# Autodesk Inventor assembly: CNC3
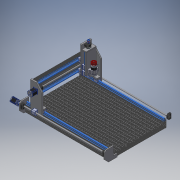
[picture p0: Inventor's stored thumbnail of the model, 180x180]
Saved by Autodesk Inventor 2018 (Build 220112000, 112)
## iProperties
Created: 2018-10-09
Part Number: CNC3
Material: Genérico
Document SubType Name: Assembly
Designer: Georgines
Author: Georgines
## Documents named in this file (29)
- C:\Users\Georgines\Documents\OpenCNC\MONTAGEM\CNC3.iam
- C:\Users\Georgines\Documents\OpenCNC\COMPONENTES_MECANICOS\BLOCOS_GUIAS_LINEARES\SBR16UU.ipt
- C:\Users\Georgines\Documents\OpenCNC\MONTAGEM\CNC1\APOIO_PERFIL_STRUTURAL.ipt
- C:\Users\Georgines\Documents\OpenCNC\MONTAGEM\CNC1\LATERAL_BLOCOS_BASE.ipt
- C:\Users\Georgines\Documents\OpenCNC\MONTAGEM\BLOCO_SUPORTE_EIXO_Z.ipt
- C:\Users\Georgines\Documents\OpenCNC\BAIXADOS\spindle-bldc-500w-1.snapshot.1\SPINDLE_500WSpindle.iam
- C:\Users\Georgines\Documents\OpenCNC\BAIXADOS\spindle-bracket-1.snapshot.2\SUPORTE_SPINDLESpindle Bracket.ipt
- C:\Users\Georgines\Documents\OpenCNC\MONTAGEM\CNC1\BLOCO_SUPORTE_SPINDLE.ipt
- C:\Users\Georgines\Documents\OpenCNC\BAIXADOS\bearing-support-unit-1.snapshot.1\BK12BK12.ipt
- C:\Users\Georgines\Documents\OpenCNC\BAIXADOS\bearing-support-unit-1.snapshot.1\BF12.ipt
- C:\Users\Georgines\Documents\OpenCNC\COMPONENTES_MECANICOS\GUIAS_LINEARES\SBR16_200MM.ipt
- C:\Users\Georgines\Documents\OpenCNC\COMPONENTES_MECANICOS\GUIAS_LINEARES\SBR16_EIXO_X_1.ipt
- C:\Users\Georgines\Documents\OpenCNC\BAIXADOS\stepper motor NEMA 23 57x76.ipt
- C:\Users\Georgines\Documents\OpenCNC\MONTAGEM\CHAPA_APOIO_CASTANHA_EIXO_Z.ipt
- C:\Users\Georgines\Documents\OpenCNC\COMPONENTES_MECANICOS\GUIAS_LINEARES\SBR16_EIXO_Y_1.ipt
- C:\Users\Georgines\Documents\OpenCNC\COMPONENTES_MECANICOS\GUIAS_LINEARES\SBR16_EIXO_Y_2.ipt
- C:\Users\Georgines\Documents\OpenCNC\COMPONENTES_MECANICOS\PERFIL_ESTRUTURAL\PERFIL_ESTRUTURAL_40X80_EIXO_Y.ipt
- C:\Users\Georgines\Documents\OpenCNC\COMPONENTES_MECANICOS\PERFIL_ESTRUTURAL\PERFIL_ESTRUTURAL_40X40_EIXO_Y_PERPENDICULAR.ipt
- C:\Users\Georgines\Documents\OpenCNC\COMPONENTES_MECANICOS\FUSOS\SFU16XX_Y1.ipt
- C:\Users\Georgines\Documents\OpenCNC\COMPONENTES_MECANICOS\FUSOS\SFU16XX_Y2.ipt
- C:\Users\Georgines\Documents\OpenCNC\COMPONENTES_MECANICOS\FUSOS\SFU16XX_Z.ipt
- C:\Users\Georgines\Documents\OpenCNC\COMPONENTES_MECANICOS\FUSOS\SFU16XX_X.ipt
- C:\Users\Georgines\Documents\OpenCNC\COMPONENTES_MECANICOS\CASTANHAS\CASTANHA_SFU1604SFU1604.ipt
- C:\Users\Georgines\Documents\OpenCNC\COMPONENTES_MECANICOS\ACOPLADORES\ACLOPLADOR_Jaw 6,35x10 d=25 L=30.ipt
- C:\Users\Georgines\Documents\OpenCNC\COMPONENTES_MECANICOS\PERFIL_ESTRUTURAL\PERFIL_ESTRUTURAL_30X60_EIXO_X1.ipt
- C:\Users\Georgines\Documents\OpenCNC\COMPONENTES_MECANICOS\PERFIL_ESTRUTURAL\PERFIL_ESTRUTURAL_30X60_EIXO_X2.ipt
- C:\Users\Georgines\Documents\OpenCNC\COMPONENTES_MECANICOS\SUPORTE_CASTANHAS\SUPORTE_CASTANHAS_DSG16H.ipt
- C:\Users\Georgines\Documents\OpenCNC\MONTAGEM\SUPORTE_MANCAL_FRONTAL.ipt
- C:\Users\Georgines\Documents\OpenCNC\COMPONENTES_MECANICOS\PERFIL_ESTRUTURAL\PERFIL_ESTRUTURAL_20X40_MESA.ipt
## Components (79 placed, 28 different names)
1. SBR16UU:1 — ALINHAMENTO_BOCOS_BASE, ALINHAMENTO_BOCOS_BASE_4, ALINHAMENTO_BOCOS_BASE_6, Alinhamento:32, Alinhamento:33, Coincidência:22, Coincidência:109
2. SBR16UU:2 — ALINHAMENTO_BOCOS_BASE_2, ALINHAMENTO_BOCOS_BASE_4, Alinhamento:31, Alinhamento:149, Coincidência:110
3. SBR16UU:3 — ALINHAMENTO_BOCOS_BASE_2, Alinhamento:81, Alinhamento:148, Coincidência:111
4. SBR16UU:4 — ALINHAMENTO_BOCOS_BASE, ALINHAMENTO_BOCOS_BASE_6, Coincidência:49, Alinhamento:82, Coincidência:108
5. APOIO_PERFIL_STRUTURAL:1 — Alinhamento:31, Alinhamento:32, Alinhamento:33, Coincidência:22, Coincidência:51, Alinhamento:85, Alinhamento:149, Alinhamento:177, Alinhamento:248
6. LATERAL_BLOCOS_BASE:1 — Alinhamento:83, Coincidência:51, Alinhamento:85, Alinhamento:177, Coincidência:173, Alinhamento:191, Alinhamento:192, Coincidência:191, Ângulo:3, Alinhamento:200, Ângulo:9, Coincidência:198, Ângulo:16, Alinhamento:208
7. BLOCO_SUPORTE_EIXO_Z:1 — Coincidência:66, Coincidência:77, Alinhamento:118, Alinhamento:122, Alinhamento:123, Alinhamento:124, Alinhamento:193, Coincidência:185, Coincidência:186, Alinhamento:196, Alinhamento:197, Coincidência:200, Alinhamento:202, Coincidência:204
8. APOIO_PERFIL_STRUTURAL:2 — Coincidência:49, Alinhamento:81, Alinhamento:82, Coincidência:52, Alinhamento:87, Alinhamento:148
9. LATERAL_BLOCOS_BASE:2 — Alinhamento:83, Coincidência:52, Alinhamento:87, Coincidência:174, Coincidência:194, Ângulo:4, Alinhamento:201, Ângulo:10, Coincidência:204
10. SPINDLE_500WSpindle:1 [sub-assembly] — Coincidência:63, Alinhamento:99
11. SUPORTE_SPINDLESpindle Bracket:1 — Coincidência:62, Alinhamento:97, Alinhamento:98, Coincidência:63, Alinhamento:99
12. BLOCO_SUPORTE_SPINDLE:1 — Coincidência:62, Alinhamento:97, Alinhamento:98, Coincidência:79, Coincidência:81, Alinhamento:119, Alinhamento:120, Alinhamento:121, Alinhamento:151, Alinhamento:152, Alinhamento:153
13. BK12BK12:1 — Coincidência:66, Alinhamento:103, Alinhamento:124, Coincidência:181, Coincidência:182, Coincidência:203
14. BF12:1 — Alinhamento:103, Alinhamento:123, Coincidência:180, Coincidência:184
15. SBR16UU:9 — Alinhamento:104, Alinhamento:106, Alinhamento:109, Coincidência:75, Coincidência:76, Coincidência:77, Coincidência:78, Alinhamento:122
16. SBR16UU:10 — Alinhamento:104, Alinhamento:107, Alinhamento:108, Alinhamento:109, Coincidência:76, Coincidência:80
17. SBR16UU:11 — Alinhamento:105, Alinhamento:106, Alinhamento:110, Coincidência:75
18. SBR16UU:12 — Alinhamento:105, Alinhamento:107, Alinhamento:108, Alinhamento:110, Alinhamento:118
19. SBR16_200MM:1 — Coincidência:78, Coincidência:79, Alinhamento:119, Alinhamento:121
20. SBR16_200MM:2 — Coincidência:80, Coincidência:81, Alinhamento:120
21. SBR16UU:13 — Coincidência:169, Alinhamento:189, Alinhamento:194, Coincidência:186, Alinhamento:197
22. SBR16UU:14 — Coincidência:168, Alinhamento:190, Alinhamento:195, Coincidência:185, Alinhamento:196
23. SBR16UU:15 — Alinhamento:173, Coincidência:166, Alinhamento:190, Alinhamento:193, Alinhamento:195
24. stepper motor NEMA 23 57x76:1 — Coincidência:187, Coincidência:188, Coincidência:198, Ângulo:12
25. CHAPA_APOIO_CASTANHA_EIXO_Z:1 — Alinhamento:151, Alinhamento:152, Alinhamento:153, Coincidência:177, Ângulo:1
26. SBR16_EIXO_Y_1:1 — Coincidência:109, Coincidência:110, Alinhamento:154, Alinhamento:157, Coincidência:115, Alinhamento:158, Alinhamento:159
27. SBR16_EIXO_Y_2:1 — Coincidência:108, Coincidência:111, Alinhamento:154, Alinhamento:157, Coincidência:116, Alinhamento:160, Alinhamento:161
28. PERFIL_ESTRUTURAL_40X80_EIXO_Y:1 — Coincidência:115, Alinhamento:158, Alinhamento:159, Alinhamento:164, Alinhamento:165, Alinhamento:166, Coincidência:131, Coincidência:133, Ângulo:9, Alinhamento:203, Alinhamento:205
29. PERFIL_ESTRUTURAL_40X80_EIXO_Y:2 — Coincidência:116, Alinhamento:160, Alinhamento:161, Coincidência:117, Alinhamento:162, Alinhamento:163, Coincidência:118, Coincidência:119, Coincidência:132, Ângulo:10, Coincidência:231
30. PERFIL_ESTRUTURAL_40X40_EIXO_Y_PERPENDICULAR:1 — Coincidência:117, Alinhamento:162, Alinhamento:163, Coincidência:210, Alinhamento:247
31. PERFIL_ESTRUTURAL_40X40_EIXO_Y_PERPENDICULAR:2 — Coincidência:118, Alinhamento:164, Alinhamento:165, Alinhamento:167
32. PERFIL_ESTRUTURAL_40X40_EIXO_Y_PERPENDICULAR:3 — Coincidência:119, Alinhamento:166, Alinhamento:167
33. stepper motor NEMA 23 57x76:3 — Coincidência:159, Coincidência:160, Ângulo:17, Ângulo:18
34. SBR16UU:17 — Alinhamento:173, Coincidência:167, Alinhamento:189, Alinhamento:194
35. SFU16XX_Y1:1 — Coincidência:136, Coincidência:137, Coincidência:138, Coincidência:139, Coincidência:152, Coincidência:155, Coincidência:157
36. SFU16XX_Y2:1 — Coincidência:140, Coincidência:141, Coincidência:142, Coincidência:143, Coincidência:153, Coincidência:156, Coincidência:158
37. SFU16XX_Z:1 — Coincidência:178, Coincidência:179, Coincidência:180, Coincidência:181, Coincidência:182, Coincidência:183, Coincidência:184
38. SFU16XX_X:1 — Coincidência:146, Coincidência:148, Coincidência:149, Coincidência:151, Coincidência:154, Coincidência:175, Coincidência:176
39. BK12BK12:2 — Coincidência:136, Coincidência:137, Alinhamento:178, Ângulo:16, Coincidência:206
40. BF12:2 — Coincidência:138, Coincidência:139, Alinhamento:178, Alinhamento:181, Alinhamento:198, Alinhamento:203, Coincidência:205
41. BK12BK12:3 — Coincidência:140, Coincidência:141, Alinhamento:179
42. BF12:3 — Coincidência:142, Coincidência:143, Alinhamento:179, Alinhamento:181, Alinhamento:198
43. BK12BK12:4 — Coincidência:146, Alinhamento:180, Coincidência:151, Ângulo:12
44. BF12:4 — Coincidência:148, Coincidência:149, Alinhamento:180, Ângulo:14, Alinhamento:212
45. CASTANHA_SFU1604SFU1604:1 — Coincidência:152, Coincidência:189, Coincidência:190, Ângulo:2
46. CASTANHA_SFU1604SFU1604:2 — Coincidência:153, Coincidência:192, Coincidência:193, Ângulo:13
47. CASTANHA_SFU1604SFU1604:3 — Coincidência:154, Coincidência:195, Coincidência:196, Ângulo:11
48. CASTANHA_SFU1604SFU1604:4 — Coincidência:177, Coincidência:178, Ângulo:1, Coincidência:203
49. ACLOPLADOR_Jaw 6,35x10 d=25 L=30:1 — Coincidência:156, Coincidência:158, Coincidência:201, Coincidência:202
50. ACLOPLADOR_Jaw 6,35x10 d=25 L=30:2 — Coincidência:155, Coincidência:157, Coincidência:159, Coincidência:160
51. ACLOPLADOR_Jaw 6,35x10 d=25 L=30:3 — Coincidência:179, Coincidência:183
52. ACLOPLADOR_Jaw 6,35x10 d=25 L=30:4 — Coincidência:175, Coincidência:176, Coincidência:187, Coincidência:188
53. PERFIL_ESTRUTURAL_30X60_EIXO_X1:1 — Coincidência:163, Alinhamento:183, Alinhamento:184, Alinhamento:187, Alinhamento:188, Coincidência:173, Alinhamento:191, Coincidência:174, Alinhamento:192, Coincidência:207, Alinhamento:209, Alinhamento:210
54. PERFIL_ESTRUTURAL_30X60_EIXO_X2:1 — Coincidência:164, Alinhamento:185, Alinhamento:186, Alinhamento:187, Alinhamento:188, Coincidência:208, Alinhamento:211
55. SBR16_EIXO_X_1:2 — Coincidência:163, Alinhamento:183, Alinhamento:184, Coincidência:168, Coincidência:169, Ângulo:14
56. SBR16_EIXO_X_1:3 — Coincidência:164, Alinhamento:185, Alinhamento:186, Coincidência:166, Coincidência:167
57. SUPORTE_CASTANHAS_DSG16H:1 — Coincidência:189, Coincidência:190, Ângulo:2, Coincidência:191, Ângulo:3, Alinhamento:200, Coincidência:205, Alinhamento:208
58. SUPORTE_CASTANHAS_DSG16H:2 — Coincidência:192, Coincidência:193, Coincidência:194, Ângulo:4, Alinhamento:201, Ângulo:13
59. SUPORTE_CASTANHAS_DSG16H:3 — Coincidência:195, Coincidência:196, Ângulo:11, Coincidência:200, Alinhamento:202
60. stepper motor NEMA 23 57x76:4 — Coincidência:201, Coincidência:202, Ângulo:17
61. SUPORTE_MANCAL_FRONTAL:1 — Alinhamento:205, Alinhamento:206, Alinhamento:207, Coincidência:211, Alinhamento:247, Alinhamento:248
62. SUPORTE_MANCAL_FRONTAL:2 — Coincidência:206, Alinhamento:206, Alinhamento:207, Ângulo:18
63. PERFIL_ESTRUTURAL_30X60_EIXO_X1:2 — Coincidência:207, Alinhamento:209, Alinhamento:210, Coincidência:208, Alinhamento:211, Alinhamento:212
64. PERFIL_ESTRUTURAL_20X40_MESA:1 — Coincidência:209, Coincidência:210, Coincidência:211, Alinhamento:213, Alinhamento:214
65. PERFIL_ESTRUTURAL_20X40_MESA:2 — Coincidência:209, Alinhamento:213, Alinhamento:214, Alinhamento:215, Alinhamento:216, Coincidência:213
66. PERFIL_ESTRUTURAL_20X40_MESA:3 — Alinhamento:215, Alinhamento:216, Coincidência:213, Coincidência:214, Alinhamento:217, Alinhamento:218
67. PERFIL_ESTRUTURAL_20X40_MESA:4 — Coincidência:214, Coincidência:215, Alinhamento:217, Alinhamento:218, Coincidência:216, Alinhamento:219, Alinhamento:220
68. PERFIL_ESTRUTURAL_20X40_MESA:5 — Coincidência:215, Coincidência:216, Alinhamento:219, Alinhamento:220, Coincidência:217, Alinhamento:221, Alinhamento:222
69. PERFIL_ESTRUTURAL_20X40_MESA:6 — Coincidência:217, Alinhamento:221, Alinhamento:222, Coincidência:218, Alinhamento:223, Alinhamento:224
70. PERFIL_ESTRUTURAL_20X40_MESA:7 — Coincidência:218, Alinhamento:223, Alinhamento:224, Coincidência:219, Alinhamento:225, Alinhamento:226
71. PERFIL_ESTRUTURAL_20X40_MESA:8 — Coincidência:219, Alinhamento:225, Alinhamento:226, Coincidência:220, Alinhamento:227, Alinhamento:228
72. PERFIL_ESTRUTURAL_20X40_MESA:9 — Coincidência:220, Alinhamento:227, Alinhamento:228, Coincidência:230, Alinhamento:245, Alinhamento:246
73. PERFIL_ESTRUTURAL_20X40_MESA:10 — Coincidência:230, Alinhamento:245, Alinhamento:246
74. PERFIL_ESTRUTURAL_20X40_MESA:11
75. PERFIL_ESTRUTURAL_20X40_MESA:12
76. PERFIL_ESTRUTURAL_20X40_MESA:13
77. PERFIL_ESTRUTURAL_20X40_MESA:14
78. PERFIL_ESTRUTURAL_20X40_MESA:15
79. PERFIL_ESTRUTURAL_20X40_MESA:16 — Coincidência:231
## Relationships (233: Flush 113, Mate 107, Angle 13)
- ALINHAMENTO_BOCOS_BASE [Flush]: SBR16UU:1 ↔ SBR16UU:4
- ALINHAMENTO_BOCOS_BASE_2 [Flush]: SBR16UU:2 ↔ SBR16UU:3
- ALINHAMENTO_BOCOS_BASE_4 [Flush]: SBR16UU:1 ↔ SBR16UU:2
- ALINHAMENTO_BOCOS_BASE_6 [Flush]: SBR16UU:1 ↔ SBR16UU:4
- Alinhamento:31 [Flush]: SBR16UU:2 ↔ APOIO_PERFIL_STRUTURAL:1
- Alinhamento:32 [Flush]: SBR16UU:1 ↔ APOIO_PERFIL_STRUTURAL:1
- Alinhamento:33 [Flush]: SBR16UU:1 ↔ APOIO_PERFIL_STRUTURAL:1
- Coincidência:22 [Mate]: SBR16UU:1 ↔ APOIO_PERFIL_STRUTURAL:1
- Coincidência:49 [Mate]: SBR16UU:4 ↔ APOIO_PERFIL_STRUTURAL:2
- Alinhamento:81 [Flush]: SBR16UU:3 ↔ APOIO_PERFIL_STRUTURAL:2
- Alinhamento:82 [Flush]: SBR16UU:4 ↔ APOIO_PERFIL_STRUTURAL:2
- Alinhamento:83 [Flush]: LATERAL_BLOCOS_BASE:1 ↔ LATERAL_BLOCOS_BASE:2
- Coincidência:51 [Mate]: APOIO_PERFIL_STRUTURAL:1 ↔ LATERAL_BLOCOS_BASE:1
- Alinhamento:85 [Flush] (-55 mm): APOIO_PERFIL_STRUTURAL:1 ↔ LATERAL_BLOCOS_BASE:1
- Coincidência:52 [Mate]: APOIO_PERFIL_STRUTURAL:2 ↔ LATERAL_BLOCOS_BASE:2
- Alinhamento:87 [Flush]: APOIO_PERFIL_STRUTURAL:2 ↔ LATERAL_BLOCOS_BASE:2
- Coincidência:62 [Mate]: SUPORTE_SPINDLESpindle Bracket:1 ↔ BLOCO_SUPORTE_SPINDLE:1
- Alinhamento:97 [Flush] (25 mm): SUPORTE_SPINDLESpindle Bracket:1 ↔ BLOCO_SUPORTE_SPINDLE:1
- Alinhamento:98 [Flush] (18 mm): SUPORTE_SPINDLESpindle Bracket:1 ↔ BLOCO_SUPORTE_SPINDLE:1
- Coincidência:63 [Mate]: SPINDLE_500WSpindle:1 ↔ SUPORTE_SPINDLESpindle Bracket:1
- Alinhamento:99 [Flush] (-25 mm): SPINDLE_500WSpindle:1 ↔ SUPORTE_SPINDLESpindle Bracket:1
- Coincidência:66 [Mate]: BLOCO_SUPORTE_EIXO_Z:1 ↔ BK12BK12:1
- Alinhamento:103 [Flush]: BK12BK12:1 ↔ BF12:1
- Alinhamento:104 [Flush]: SBR16UU:9 ↔ SBR16UU:10
- Alinhamento:105 [Flush]: SBR16UU:11 ↔ SBR16UU:12
- Alinhamento:106 [Flush]: SBR16UU:9 ↔ SBR16UU:11
- Alinhamento:107 [Flush]: SBR16UU:10 ↔ SBR16UU:12
- Alinhamento:108 [Flush]: SBR16UU:10 ↔ SBR16UU:12
- Alinhamento:109 [Flush]: SBR16UU:9 ↔ SBR16UU:10
- Alinhamento:110 [Flush]: SBR16UU:11 ↔ SBR16UU:12
- Coincidência:75 [Mate] (23 mm): SBR16UU:9 ↔ SBR16UU:11
- Coincidência:76 [Mate] (35 mm): SBR16UU:9 ↔ SBR16UU:10
- Coincidência:77 [Mate]: BLOCO_SUPORTE_EIXO_Z:1 ↔ SBR16UU:9
- Alinhamento:118 [Flush]: BLOCO_SUPORTE_EIXO_Z:1 ↔ SBR16UU:12
- Coincidência:78 [Mate]: SBR16UU:9 ↔ SBR16_200MM:1
- Coincidência:79 [Mate]: BLOCO_SUPORTE_SPINDLE:1 ↔ SBR16_200MM:1
- Coincidência:80 [Mate]: SBR16UU:10 ↔ SBR16_200MM:2
- Coincidência:81 [Mate]: BLOCO_SUPORTE_SPINDLE:1 ↔ SBR16_200MM:2
- Alinhamento:119 [Flush]: BLOCO_SUPORTE_SPINDLE:1 ↔ SBR16_200MM:1
- Alinhamento:120 [Flush]: BLOCO_SUPORTE_SPINDLE:1 ↔ SBR16_200MM:2
- Alinhamento:121 [Flush] (-2.5 mm): BLOCO_SUPORTE_SPINDLE:1 ↔ SBR16_200MM:1
- Alinhamento:122 [Flush]: BLOCO_SUPORTE_EIXO_Z:1 ↔ SBR16UU:9
- Alinhamento:123 [Flush] (46.627 mm): BLOCO_SUPORTE_EIXO_Z:1 ↔ BF12:1
- Alinhamento:124 [Flush] (32.5 mm): BLOCO_SUPORTE_EIXO_Z:1 ↔ BK12BK12:1
- Alinhamento:148 [Flush]: SBR16UU:3 ↔ APOIO_PERFIL_STRUTURAL:2
- Alinhamento:149 [Flush]: SBR16UU:2 ↔ APOIO_PERFIL_STRUTURAL:1
- Alinhamento:151 [Flush]: BLOCO_SUPORTE_SPINDLE:1 ↔ CHAPA_APOIO_CASTANHA_EIXO_Z:1
- Alinhamento:152 [Flush]: BLOCO_SUPORTE_SPINDLE:1 ↔ CHAPA_APOIO_CASTANHA_EIXO_Z:1
- Alinhamento:153 [Flush]: BLOCO_SUPORTE_SPINDLE:1 ↔ CHAPA_APOIO_CASTANHA_EIXO_Z:1
- Coincidência:108 [Mate]: SBR16UU:4 ↔ SBR16_EIXO_Y_2:1
- Coincidência:109 [Mate]: SBR16UU:1 ↔ SBR16_EIXO_Y_1:1
- Coincidência:110 [Mate]: SBR16UU:2 ↔ SBR16_EIXO_Y_1:1
- Coincidência:111 [Mate]: SBR16UU:3 ↔ SBR16_EIXO_Y_2:1
- Alinhamento:154 [Flush]: SBR16_EIXO_Y_1:1 ↔ SBR16_EIXO_Y_2:1
- Alinhamento:157 [Flush]: SBR16_EIXO_Y_1:1 ↔ SBR16_EIXO_Y_2:1
- Coincidência:115 [Mate]: SBR16_EIXO_Y_1:1 ↔ PERFIL_ESTRUTURAL_40X80_EIXO_Y:1
- Coincidência:116 [Mate]: SBR16_EIXO_Y_2:1 ↔ PERFIL_ESTRUTURAL_40X80_EIXO_Y:2
- Alinhamento:158 [Flush]: SBR16_EIXO_Y_1:1 ↔ PERFIL_ESTRUTURAL_40X80_EIXO_Y:1
- Alinhamento:159 [Flush]: SBR16_EIXO_Y_1:1 ↔ PERFIL_ESTRUTURAL_40X80_EIXO_Y:1
- Alinhamento:160 [Flush]: SBR16_EIXO_Y_2:1 ↔ PERFIL_ESTRUTURAL_40X80_EIXO_Y:2
- Alinhamento:161 [Flush]: SBR16_EIXO_Y_2:1 ↔ PERFIL_ESTRUTURAL_40X80_EIXO_Y:2
- Coincidência:117 [Mate]: PERFIL_ESTRUTURAL_40X80_EIXO_Y:2 ↔ PERFIL_ESTRUTURAL_40X40_EIXO_Y_PERPENDICULAR:1
- Alinhamento:162 [Flush]: PERFIL_ESTRUTURAL_40X80_EIXO_Y:2 ↔ PERFIL_ESTRUTURAL_40X40_EIXO_Y_PERPENDICULAR:1
- Alinhamento:163 [Flush]: PERFIL_ESTRUTURAL_40X80_EIXO_Y:2 ↔ PERFIL_ESTRUTURAL_40X40_EIXO_Y_PERPENDICULAR:1
- Coincidência:118 [Mate]: PERFIL_ESTRUTURAL_40X80_EIXO_Y:2 ↔ PERFIL_ESTRUTURAL_40X40_EIXO_Y_PERPENDICULAR:2
- Alinhamento:164 [Flush]: PERFIL_ESTRUTURAL_40X80_EIXO_Y:1 ↔ PERFIL_ESTRUTURAL_40X40_EIXO_Y_PERPENDICULAR:2
- Alinhamento:165 [Flush]: PERFIL_ESTRUTURAL_40X80_EIXO_Y:1 ↔ PERFIL_ESTRUTURAL_40X40_EIXO_Y_PERPENDICULAR:2
- Coincidência:119 [Mate]: PERFIL_ESTRUTURAL_40X80_EIXO_Y:2 ↔ PERFIL_ESTRUTURAL_40X40_EIXO_Y_PERPENDICULAR:3
- Alinhamento:166 [Flush]: PERFIL_ESTRUTURAL_40X80_EIXO_Y:1 ↔ PERFIL_ESTRUTURAL_40X40_EIXO_Y_PERPENDICULAR:3
- Alinhamento:167 [Flush] (-433.419 mm): PERFIL_ESTRUTURAL_40X40_EIXO_Y_PERPENDICULAR:2 ↔ PERFIL_ESTRUTURAL_40X40_EIXO_Y_PERPENDICULAR:3
- Alinhamento:173 [Flush]: SBR16UU:15 ↔ SBR16UU:17
- Coincidência:131 [Mate]: PERFIL_ESTRUTURAL_40X80_EIXO_Y:1
- Coincidência:132 [Mate]: PERFIL_ESTRUTURAL_40X80_EIXO_Y:2
- Coincidência:133 [Mate]: PERFIL_ESTRUTURAL_40X80_EIXO_Y:1
- Alinhamento:177 [Flush]: APOIO_PERFIL_STRUTURAL:1 ↔ LATERAL_BLOCOS_BASE:1
- Coincidência:136 [Mate]: SFU16XX_Y1:1 ↔ BK12BK12:2
- Coincidência:137 [Mate]: SFU16XX_Y1:1 ↔ BK12BK12:2
- Coincidência:138 [Mate]: SFU16XX_Y1:1 ↔ BF12:2
- Coincidência:139 [Mate]: SFU16XX_Y1:1 ↔ BF12:2
- Coincidência:140 [Mate]: SFU16XX_Y2:1 ↔ BK12BK12:3
- Coincidência:141 [Mate]: SFU16XX_Y2:1 ↔ BK12BK12:3
- Coincidência:142 [Mate]: SFU16XX_Y2:1 ↔ BF12:3
- Coincidência:143 [Mate]: SFU16XX_Y2:1 ↔ BF12:3
- Alinhamento:178 [Flush]: BK12BK12:2 ↔ BF12:2
- Alinhamento:179 [Flush]: BK12BK12:3 ↔ BF12:3
- Coincidência:146 [Mate]: SFU16XX_X:1 ↔ BK12BK12:4
- Coincidência:148 [Mate]: SFU16XX_X:1 ↔ BF12:4
- Coincidência:149 [Mate]: SFU16XX_X:1 ↔ BF12:4
- Alinhamento:180 [Flush]: BK12BK12:4 ↔ BF12:4
- Coincidência:151 [Mate]: SFU16XX_X:1 ↔ BK12BK12:4
- Coincidência:152 [Mate]: SFU16XX_Y1:1 ↔ CASTANHA_SFU1604SFU1604:1
- Coincidência:153 [Mate]: SFU16XX_Y2:1 ↔ CASTANHA_SFU1604SFU1604:2
- Coincidência:154 [Mate]: SFU16XX_X:1 ↔ CASTANHA_SFU1604SFU1604:3
- Coincidência:155 [Mate]: SFU16XX_Y1:1 ↔ ACLOPLADOR_Jaw 6,35x10 d=25 L=30:2
- Coincidência:156 [Mate]: SFU16XX_Y2:1 ↔ ACLOPLADOR_Jaw 6,35x10 d=25 L=30:1
- Coincidência:157 [Mate]: SFU16XX_Y1:1 ↔ ACLOPLADOR_Jaw 6,35x10 d=25 L=30:2
- Coincidência:158 [Mate]: SFU16XX_Y2:1 ↔ ACLOPLADOR_Jaw 6,35x10 d=25 L=30:1
- Alinhamento:181 [Flush]: BF12:2 ↔ BF12:3
- Coincidência:159 [Mate]: stepper motor NEMA 23 57x76:3 ↔ ACLOPLADOR_Jaw 6,35x10 d=25 L=30:2
- Coincidência:160 [Mate] (-15 mm): stepper motor NEMA 23 57x76:3 ↔ ACLOPLADOR_Jaw 6,35x10 d=25 L=30:2
- Coincidência:163 [Mate]: PERFIL_ESTRUTURAL_30X60_EIXO_X1:1 ↔ SBR16_EIXO_X_1:2
- Alinhamento:183 [Flush]: PERFIL_ESTRUTURAL_30X60_EIXO_X1:1 ↔ SBR16_EIXO_X_1:2
- Alinhamento:184 [Flush] (-10 mm): PERFIL_ESTRUTURAL_30X60_EIXO_X1:1 ↔ SBR16_EIXO_X_1:2
- Coincidência:164 [Mate]: PERFIL_ESTRUTURAL_30X60_EIXO_X2:1 ↔ SBR16_EIXO_X_1:3
- Alinhamento:185 [Flush]: PERFIL_ESTRUTURAL_30X60_EIXO_X2:1 ↔ SBR16_EIXO_X_1:3
- Alinhamento:186 [Flush] (10 mm): PERFIL_ESTRUTURAL_30X60_EIXO_X2:1 ↔ SBR16_EIXO_X_1:3
- Alinhamento:187 [Flush]: PERFIL_ESTRUTURAL_30X60_EIXO_X1:1 ↔ PERFIL_ESTRUTURAL_30X60_EIXO_X2:1
- Alinhamento:188 [Flush]: PERFIL_ESTRUTURAL_30X60_EIXO_X1:1 ↔ PERFIL_ESTRUTURAL_30X60_EIXO_X2:1
- Coincidência:166 [Mate]: SBR16UU:15 ↔ SBR16_EIXO_X_1:3
- Coincidência:167 [Mate]: SBR16UU:17 ↔ SBR16_EIXO_X_1:3
- Coincidência:168 [Mate]: SBR16UU:14 ↔ SBR16_EIXO_X_1:2
- Coincidência:169 [Mate]: SBR16UU:13 ↔ SBR16_EIXO_X_1:2
- Alinhamento:189 [Flush]: SBR16UU:13 ↔ SBR16UU:17
- Alinhamento:190 [Flush]: SBR16UU:14 ↔ SBR16UU:15
- Coincidência:173 [Mate]: LATERAL_BLOCOS_BASE:1 ↔ PERFIL_ESTRUTURAL_30X60_EIXO_X1:1
- Alinhamento:191 [Flush] (10 mm): LATERAL_BLOCOS_BASE:1 ↔ PERFIL_ESTRUTURAL_30X60_EIXO_X1:1
- Coincidência:174 [Mate]: LATERAL_BLOCOS_BASE:2 ↔ PERFIL_ESTRUTURAL_30X60_EIXO_X1:1
- Alinhamento:192 [Flush]: LATERAL_BLOCOS_BASE:1 ↔ PERFIL_ESTRUTURAL_30X60_EIXO_X1:1
- Alinhamento:193 [Flush]: BLOCO_SUPORTE_EIXO_Z:1 ↔ SBR16UU:15
- Coincidência:175 [Mate]: SFU16XX_X:1 ↔ ACLOPLADOR_Jaw 6,35x10 d=25 L=30:4
- Coincidência:176 [Mate] (-15 mm): SFU16XX_X:1 ↔ ACLOPLADOR_Jaw 6,35x10 d=25 L=30:4
- Coincidência:177 [Mate]: CHAPA_APOIO_CASTANHA_EIXO_Z:1 ↔ CASTANHA_SFU1604SFU1604:4
- Coincidência:178 [Mate]: SFU16XX_Z:1 ↔ CASTANHA_SFU1604SFU1604:4
- Coincidência:179 [Mate]: SFU16XX_Z:1 ↔ ACLOPLADOR_Jaw 6,35x10 d=25 L=30:3
- Coincidência:180 [Mate]: BF12:1 ↔ SFU16XX_Z:1
- Coincidência:181 [Mate]: BK12BK12:1 ↔ SFU16XX_Z:1
- Coincidência:182 [Mate]: BK12BK12:1 ↔ SFU16XX_Z:1
- Ângulo:1 [Angle] (0 deg): CHAPA_APOIO_CASTANHA_EIXO_Z:1 ↔ CASTANHA_SFU1604SFU1604:4
- Coincidência:183 [Mate] (-15 mm): SFU16XX_Z:1 ↔ ACLOPLADOR_Jaw 6,35x10 d=25 L=30:3
- Coincidência:184 [Mate]: BF12:1 ↔ SFU16XX_Z:1
- Alinhamento:194 [Flush]: SBR16UU:13 ↔ SBR16UU:17
- Alinhamento:195 [Flush]: SBR16UU:14 ↔ SBR16UU:15
- Coincidência:185 [Mate]: BLOCO_SUPORTE_EIXO_Z:1 ↔ SBR16UU:14
- Coincidência:186 [Mate]: BLOCO_SUPORTE_EIXO_Z:1 ↔ SBR16UU:13
- Alinhamento:196 [Flush]: BLOCO_SUPORTE_EIXO_Z:1 ↔ SBR16UU:14
- Alinhamento:197 [Flush]: BLOCO_SUPORTE_EIXO_Z:1 ↔ SBR16UU:13
- Coincidência:187 [Mate]: stepper motor NEMA 23 57x76:1 ↔ ACLOPLADOR_Jaw 6,35x10 d=25 L=30:4
- Coincidência:188 [Mate] (-15 mm): stepper motor NEMA 23 57x76:1 ↔ ACLOPLADOR_Jaw 6,35x10 d=25 L=30:4
- Alinhamento:198 [Flush]: BF12:2 ↔ BF12:3
- Coincidência:189 [Mate]: CASTANHA_SFU1604SFU1604:1 ↔ SUPORTE_CASTANHAS_DSG16H:1
- Coincidência:190 [Mate]: CASTANHA_SFU1604SFU1604:1 ↔ SUPORTE_CASTANHAS_DSG16H:1
- Ângulo:2 [Angle] (0 deg): CASTANHA_SFU1604SFU1604:1 ↔ SUPORTE_CASTANHAS_DSG16H:1
- Coincidência:191 [Mate]: LATERAL_BLOCOS_BASE:1 ↔ SUPORTE_CASTANHAS_DSG16H:1
- Ângulo:3 [Angle] (0 deg): LATERAL_BLOCOS_BASE:1 ↔ SUPORTE_CASTANHAS_DSG16H:1
- Coincidência:192 [Mate]: CASTANHA_SFU1604SFU1604:2 ↔ SUPORTE_CASTANHAS_DSG16H:2
- Coincidência:193 [Mate]: CASTANHA_SFU1604SFU1604:2 ↔ SUPORTE_CASTANHAS_DSG16H:2
- Coincidência:194 [Mate]: LATERAL_BLOCOS_BASE:2 ↔ SUPORTE_CASTANHAS_DSG16H:2
- Ângulo:4 [Angle] (0 deg): LATERAL_BLOCOS_BASE:2 ↔ SUPORTE_CASTANHAS_DSG16H:2
- Alinhamento:200 [Flush] (-50 mm): LATERAL_BLOCOS_BASE:1 ↔ SUPORTE_CASTANHAS_DSG16H:1
- Alinhamento:201 [Flush] (50 mm): LATERAL_BLOCOS_BASE:2 ↔ SUPORTE_CASTANHAS_DSG16H:2
- Ângulo:9 [Angle] (0 deg): LATERAL_BLOCOS_BASE:1 ↔ PERFIL_ESTRUTURAL_40X80_EIXO_Y:1
- Ângulo:10 [Angle] (0 deg): LATERAL_BLOCOS_BASE:2 ↔ PERFIL_ESTRUTURAL_40X80_EIXO_Y:2
- Coincidência:195 [Mate]: CASTANHA_SFU1604SFU1604:3 ↔ SUPORTE_CASTANHAS_DSG16H:3
- Coincidência:196 [Mate]: CASTANHA_SFU1604SFU1604:3 ↔ SUPORTE_CASTANHAS_DSG16H:3
- Ângulo:11 [Angle] (0 deg): CASTANHA_SFU1604SFU1604:3 ↔ SUPORTE_CASTANHAS_DSG16H:3
- Coincidência:198 [Mate]: LATERAL_BLOCOS_BASE:1 ↔ stepper motor NEMA 23 57x76:1
- Coincidência:200 [Mate]: BLOCO_SUPORTE_EIXO_Z:1 ↔ SUPORTE_CASTANHAS_DSG16H:3
- Ângulo:12 [Angle] (0 deg): stepper motor NEMA 23 57x76:1 ↔ BK12BK12:4
- Alinhamento:202 [Flush] (42.5 mm): BLOCO_SUPORTE_EIXO_Z:1 ↔ SUPORTE_CASTANHAS_DSG16H:3
- Ângulo:13 [Angle] (0 deg): CASTANHA_SFU1604SFU1604:2 ↔ SUPORTE_CASTANHAS_DSG16H:2
- Ângulo:14 [Angle] (0 deg): BF12:4 ↔ SBR16_EIXO_X_1:2
- Coincidência:201 [Mate]: ACLOPLADOR_Jaw 6,35x10 d=25 L=30:1 ↔ stepper motor NEMA 23 57x76:4
- Coincidência:202 [Mate] (-15 mm): ACLOPLADOR_Jaw 6,35x10 d=25 L=30:1 ↔ stepper motor NEMA 23 57x76:4
- Coincidência:203 [Mate] (155 mm): BK12BK12:1 ↔ CASTANHA_SFU1604SFU1604:4
- Coincidência:204 [Mate]: BLOCO_SUPORTE_EIXO_Z:1 ↔ LATERAL_BLOCOS_BASE:2
- Alinhamento:203 [Flush]: PERFIL_ESTRUTURAL_40X80_EIXO_Y:1 ↔ BF12:2
- Coincidência:205 [Mate]: BF12:2 ↔ SUPORTE_CASTANHAS_DSG16H:1
- Ângulo:16 [Angle] (0 deg): LATERAL_BLOCOS_BASE:1 ↔ BK12BK12:2
- Alinhamento:205 [Flush]: PERFIL_ESTRUTURAL_40X80_EIXO_Y:1 ↔ SUPORTE_MANCAL_FRONTAL:1
- Coincidência:206 [Mate]: BK12BK12:2 ↔ SUPORTE_MANCAL_FRONTAL:2
- Alinhamento:206 [Flush]: SUPORTE_MANCAL_FRONTAL:1 ↔ SUPORTE_MANCAL_FRONTAL:2
- Alinhamento:207 [Flush]: SUPORTE_MANCAL_FRONTAL:1 ↔ SUPORTE_MANCAL_FRONTAL:2
- Alinhamento:208 [Flush]: LATERAL_BLOCOS_BASE:1 ↔ SUPORTE_CASTANHAS_DSG16H:1
- Ângulo:17 [Angle] (0 deg): stepper motor NEMA 23 57x76:3 ↔ stepper motor NEMA 23 57x76:4
- Ângulo:18 [Angle] (45 deg): stepper motor NEMA 23 57x76:3 ↔ SUPORTE_MANCAL_FRONTAL:2
- Coincidência:207 [Mate]: PERFIL_ESTRUTURAL_30X60_EIXO_X1:1 ↔ PERFIL_ESTRUTURAL_30X60_EIXO_X1:2
- Alinhamento:209 [Flush]: PERFIL_ESTRUTURAL_30X60_EIXO_X1:1 ↔ PERFIL_ESTRUTURAL_30X60_EIXO_X1:2
- Alinhamento:210 [Flush]: PERFIL_ESTRUTURAL_30X60_EIXO_X1:1 ↔ PERFIL_ESTRUTURAL_30X60_EIXO_X1:2
- Coincidência:208 [Mate]: PERFIL_ESTRUTURAL_30X60_EIXO_X2:1 ↔ PERFIL_ESTRUTURAL_30X60_EIXO_X1:2
- Alinhamento:211 [Flush]: PERFIL_ESTRUTURAL_30X60_EIXO_X2:1 ↔ PERFIL_ESTRUTURAL_30X60_EIXO_X1:2
- Alinhamento:212 [Flush]: BF12:4 ↔ PERFIL_ESTRUTURAL_30X60_EIXO_X1:2
- Coincidência:209 [Mate]: PERFIL_ESTRUTURAL_20X40_MESA:1 ↔ PERFIL_ESTRUTURAL_20X40_MESA:2
- Coincidência:210 [Mate]: PERFIL_ESTRUTURAL_40X40_EIXO_Y_PERPENDICULAR:1 ↔ PERFIL_ESTRUTURAL_20X40_MESA:1
- Coincidência:211 [Mate]: SUPORTE_MANCAL_FRONTAL:1 ↔ PERFIL_ESTRUTURAL_20X40_MESA:1
- Alinhamento:213 [Flush]: PERFIL_ESTRUTURAL_20X40_MESA:1 ↔ PERFIL_ESTRUTURAL_20X40_MESA:2
- Alinhamento:214 [Flush]: PERFIL_ESTRUTURAL_20X40_MESA:1 ↔ PERFIL_ESTRUTURAL_20X40_MESA:2
- Alinhamento:215 [Flush]: PERFIL_ESTRUTURAL_20X40_MESA:2 ↔ PERFIL_ESTRUTURAL_20X40_MESA:3
- Alinhamento:216 [Flush]: PERFIL_ESTRUTURAL_20X40_MESA:2 ↔ PERFIL_ESTRUTURAL_20X40_MESA:3
- Coincidência:213 [Mate]: PERFIL_ESTRUTURAL_20X40_MESA:2 ↔ PERFIL_ESTRUTURAL_20X40_MESA:3
- Coincidência:214 [Mate]: PERFIL_ESTRUTURAL_20X40_MESA:3 ↔ PERFIL_ESTRUTURAL_20X40_MESA:4
- Coincidência:215 [Mate]: PERFIL_ESTRUTURAL_20X40_MESA:4 ↔ PERFIL_ESTRUTURAL_20X40_MESA:5
- Alinhamento:217 [Flush]: PERFIL_ESTRUTURAL_20X40_MESA:3 ↔ PERFIL_ESTRUTURAL_20X40_MESA:4
- Alinhamento:218 [Flush]: PERFIL_ESTRUTURAL_20X40_MESA:3 ↔ PERFIL_ESTRUTURAL_20X40_MESA:4
- Coincidência:216 [Mate]: PERFIL_ESTRUTURAL_20X40_MESA:4 ↔ PERFIL_ESTRUTURAL_20X40_MESA:5
- Alinhamento:219 [Flush]: PERFIL_ESTRUTURAL_20X40_MESA:4 ↔ PERFIL_ESTRUTURAL_20X40_MESA:5
- Alinhamento:220 [Flush]: PERFIL_ESTRUTURAL_20X40_MESA:4 ↔ PERFIL_ESTRUTURAL_20X40_MESA:5
- Coincidência:217 [Mate]: PERFIL_ESTRUTURAL_20X40_MESA:5 ↔ PERFIL_ESTRUTURAL_20X40_MESA:6
- Alinhamento:221 [Flush]: PERFIL_ESTRUTURAL_20X40_MESA:5 ↔ PERFIL_ESTRUTURAL_20X40_MESA:6
- Alinhamento:222 [Flush]: PERFIL_ESTRUTURAL_20X40_MESA:5 ↔ PERFIL_ESTRUTURAL_20X40_MESA:6
- Coincidência:218 [Mate]: PERFIL_ESTRUTURAL_20X40_MESA:6 ↔ PERFIL_ESTRUTURAL_20X40_MESA:7
- Alinhamento:223 [Flush]: PERFIL_ESTRUTURAL_20X40_MESA:6 ↔ PERFIL_ESTRUTURAL_20X40_MESA:7
- Alinhamento:224 [Flush]: PERFIL_ESTRUTURAL_20X40_MESA:6 ↔ PERFIL_ESTRUTURAL_20X40_MESA:7
- Coincidência:219 [Mate]: PERFIL_ESTRUTURAL_20X40_MESA:7 ↔ PERFIL_ESTRUTURAL_20X40_MESA:8
- Alinhamento:225 [Flush]: PERFIL_ESTRUTURAL_20X40_MESA:7 ↔ PERFIL_ESTRUTURAL_20X40_MESA:8
- Alinhamento:226 [Flush]: PERFIL_ESTRUTURAL_20X40_MESA:7 ↔ PERFIL_ESTRUTURAL_20X40_MESA:8
- Coincidência:220 [Mate]: PERFIL_ESTRUTURAL_20X40_MESA:8 ↔ PERFIL_ESTRUTURAL_20X40_MESA:9
- Alinhamento:227 [Flush]: PERFIL_ESTRUTURAL_20X40_MESA:8 ↔ PERFIL_ESTRUTURAL_20X40_MESA:9
- Alinhamento:228 [Flush]: PERFIL_ESTRUTURAL_20X40_MESA:8 ↔ PERFIL_ESTRUTURAL_20X40_MESA:9
- [Mate]: PERFIL_ESTRUTURAL_20X40_MESA:10 ↔ PERFIL_ESTRUTURAL_20X40_MESA:11
- [Flush]: PERFIL_ESTRUTURAL_20X40_MESA:10 ↔ PERFIL_ESTRUTURAL_20X40_MESA:11
- [Flush]: PERFIL_ESTRUTURAL_20X40_MESA:10 ↔ PERFIL_ESTRUTURAL_20X40_MESA:11
- [Flush]: PERFIL_ESTRUTURAL_20X40_MESA:11 ↔ PERFIL_ESTRUTURAL_20X40_MESA:12
- [Flush]: PERFIL_ESTRUTURAL_20X40_MESA:11 ↔ PERFIL_ESTRUTURAL_20X40_MESA:12
- [Mate]: PERFIL_ESTRUTURAL_20X40_MESA:11 ↔ PERFIL_ESTRUTURAL_20X40_MESA:12
- [Mate]: PERFIL_ESTRUTURAL_20X40_MESA:12 ↔ PERFIL_ESTRUTURAL_20X40_MESA:13
- [Mate]: PERFIL_ESTRUTURAL_20X40_MESA:13 ↔ PERFIL_ESTRUTURAL_20X40_MESA:14
- [Flush]: PERFIL_ESTRUTURAL_20X40_MESA:12 ↔ PERFIL_ESTRUTURAL_20X40_MESA:13
- [Flush]: PERFIL_ESTRUTURAL_20X40_MESA:12 ↔ PERFIL_ESTRUTURAL_20X40_MESA:13
- [Mate]: PERFIL_ESTRUTURAL_20X40_MESA:13 ↔ PERFIL_ESTRUTURAL_20X40_MESA:14
- [Flush]: PERFIL_ESTRUTURAL_20X40_MESA:13 ↔ PERFIL_ESTRUTURAL_20X40_MESA:14
- [Flush]: PERFIL_ESTRUTURAL_20X40_MESA:13 ↔ PERFIL_ESTRUTURAL_20X40_MESA:14
- [Mate]: PERFIL_ESTRUTURAL_20X40_MESA:14 ↔ PERFIL_ESTRUTURAL_20X40_MESA:15
- [Flush]: PERFIL_ESTRUTURAL_20X40_MESA:14 ↔ PERFIL_ESTRUTURAL_20X40_MESA:15
- [Flush]: PERFIL_ESTRUTURAL_20X40_MESA:14 ↔ PERFIL_ESTRUTURAL_20X40_MESA:15
- [Mate]: PERFIL_ESTRUTURAL_20X40_MESA:15 ↔ PERFIL_ESTRUTURAL_20X40_MESA:16
- [Flush]: PERFIL_ESTRUTURAL_20X40_MESA:15 ↔ PERFIL_ESTRUTURAL_20X40_MESA:16
- [Flush]: PERFIL_ESTRUTURAL_20X40_MESA:15 ↔ PERFIL_ESTRUTURAL_20X40_MESA:16
- Coincidência:230 [Mate]: PERFIL_ESTRUTURAL_20X40_MESA:9 ↔ PERFIL_ESTRUTURAL_20X40_MESA:10
- Alinhamento:245 [Flush]: PERFIL_ESTRUTURAL_20X40_MESA:9 ↔ PERFIL_ESTRUTURAL_20X40_MESA:10
- Alinhamento:246 [Flush]: PERFIL_ESTRUTURAL_20X40_MESA:9 ↔ PERFIL_ESTRUTURAL_20X40_MESA:10
- Coincidência:231 [Mate]: PERFIL_ESTRUTURAL_40X80_EIXO_Y:2 ↔ PERFIL_ESTRUTURAL_20X40_MESA:16
- Alinhamento:247 [Flush]: PERFIL_ESTRUTURAL_40X40_EIXO_Y_PERPENDICULAR:1 ↔ SUPORTE_MANCAL_FRONTAL:1
- Alinhamento:248 [Flush] (2 mm): APOIO_PERFIL_STRUTURAL:1 ↔ SUPORTE_MANCAL_FRONTAL:1
## Named parameters: d552_d524 = 0 mm, d553_d528 = 0 mm, d554_d543 = 0 mm, d555_d544 = 0 mm, d556_d545 = 0 mm, d563_d529 = 0 mm, d564_d530 = 0 mm, d565_d531 = 0 mm, d566_d532 = 0 mm, d567_d533 = 0 mm, d568_d534 = 0 mm, d569_d535 = 0 mm, d570_d536 = 0 mm, d571_d537 = 0 mm, d572_d538 = 0 mm, d573_d539 = 0 mm, d574_d540 = 0 mm, d575_d541 = 0 mm, d576_d542 = 0 mm
